# Autodesk Inventor assembly: jumper_completo
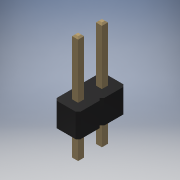
[picture p0: Inventor's stored thumbnail of the model, 180x180]
Saved by Autodesk Inventor 2019 (Build 230136000, 136)
## iProperties
Created: 2019-03-13
Part Number: jumper_completo
Material: Generico
Document SubType Name: Assembly
Designer: Thartarus
Author: Thartarus
## Documents named in this file (2)
- D:\KiCad eda\progetti kicad\SAE_Fenice\BMS_HV\CellsBoard\v2.1.1\modules\packages3d\jumper_completo.iam
- D:\KiCad eda\progetti kicad\SAE_Fenice\BMS_HV\CellsBoard\v2.1.1\modules\packages3d\jumper.ipt
## Components (1 placed, 1 different names)
1. jumper:1 — Coincidente:1, Coincidente:2, Coincidente:3
## Relationships (3: Mate 3)
- Coincidente:1 [Mate]: jumper:1
- Coincidente:2 [Mate] (-0.32 mm): jumper:1
- Coincidente:3 [Mate] (-0.32 mm): jumper:1
